# Autodesk Inventor assembly: NewTail(final)
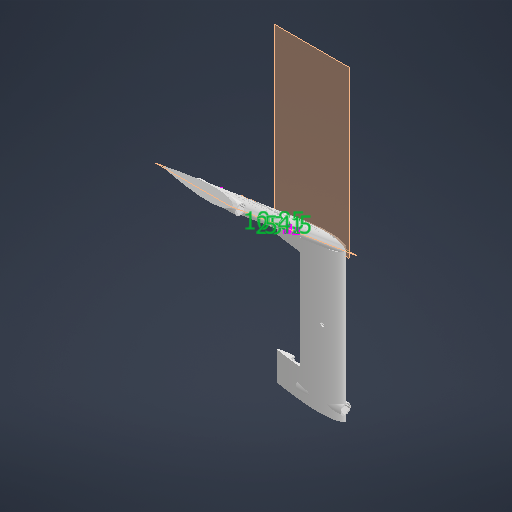
[picture p0: Inventor's stored thumbnail of the model, 512x512]
Saved by Autodesk Inventor 2026 (Build 300175050, 175E)
## iProperties
Created: 2026-08-04
Part Number: NewTail(final)
Document SubType Name: Assembly
Designer: Delbe
Author: Delbe
## Documents named in this file (5)
- C:\GitHub\SWIFT-UAV\System_development\Pelican\structural_model\v0.3.0\Parts\Delb_Parts\NewTail(final).iam
- C:\GitHub\SWIFT-UAV\System_development\Pelican\structural_model\v0.3.0\Parts\Delb_Parts\Male_Tail_Male_Connector.ipt
- C:\GitHub\SWIFT-UAV\System_development\Pelican\structural_model\v0.3.0\Parts\Delb_Parts\Female_Tail_Female_Connector.ipt
- C:\GitHub\SWIFT-UAV\System_development\Pelican\structural_model\v0.3.0\Parts\Delb_Parts\Female_Tail_Male_Connector.ipt
- C:\GitHub\SWIFT-UAV\System_development\Pelican\structural_model\v0.3.0\Parts\Delb_Parts\Male_Tail_Female_Connector(final).iam
## Components (4 placed, 4 different names)
1. Male_Tail_Male_Connector:1 — Rigid:1
2. Female_Tail_Female_Connector:1 — Mate:1, Mate:2
3. Female_Tail_Male_Connector:1 — Mate:1
4. Male_Tail_Female_Connector(final):1 [sub-assembly] — Mate:2, Rigid:1
## Relationships (3: Mate 2, WeldJoint 1)
- Mate:1: Female_Tail_Female_Connector:1 ↔ Female_Tail_Male_Connector:1
- Mate:2: Female_Tail_Female_Connector:1 ↔ Male_Tail_Female_Connector(final):1
- Rigid:1 [WeldJoint]: Male_Tail_Male_Connector:1 ↔ Male_Tail_Female_Connector(final):1
